# Autodesk Inventor assembly: Front_Train
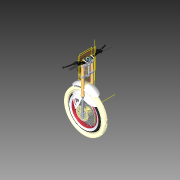
[picture p0: Inventor's stored thumbnail of the model, 180x180]
Saved by Autodesk Inventor 2016 (Build 200138000, 138)
## iProperties
Created: 2015-04-04
Part Number: Front_Train
Document SubType Name: Assembly
Designer: Yann
Author: Yann
## iProperties of the stored document Handlebar.ipt
Created: 2014-11-08
Part Number: Handlebar
Material: Generic
Document SubType Name: Modeling
Designer: Yann
Density: 1 g/cm^3
Appearance: Default
Sending System: SolidWorks 2012
Last Author: Stormtrooper
Last Saved: 2014-11-19
Author: Yann
## Documents named in this file (11)
- **C:\Users\Yann\Documents\GitHub\BIKAIR_CAD\Source\Front_Train\Front_Train.iam*LocalDocs*xOqdabbqfCq0wujc0Oz4mrtfs3b*Handlebar.ipt
- C:\Users\Yann\Documents\GitHub\BIKAIR_CAD\Source\Front_Train\Front_Train.iam
- C:\Users\Yann\Documents\GitHub\BIKAIR_CAD\Source\Front_Train\Fork\Scaled_CR85_Fork.ipt
- C:\Users\Yann\Documents\GitHub\BIKAIR_CAD\Source\Front_Train\Wheel_spokes\Wheel_spokes.iam
- C:\Users\Yann\Documents\GitHub\BIKAIR_CAD\Source\Front_Train\Headlight.iam
- C:\Users\Yann\Documents\GitHub\BIKAIR_CAD\Source\Front_Train\Front_fender.ipt
- C:\Users\Yann\Documents\GitHub\BIKAIR_CAD\Source\Front_Train\Front_fender_without_sides.ipt
- C:\Users\Yann\Documents\GitHub\BIKAIR_CAD\Source\Front_Train\Dashboard\Samsung_S5.ipt
- C:\Users\Yann\Documents\GitHub\BIKAIR_CAD\Source\Front_Train\Brakes\Levers\Manilla.iam
- C:\Users\Yann\Documents\GitHub\BIKAIR_CAD\Source\Front_Train\Handlebar_Grip.ipt
- C:\Users\Yann\Documents\GitHub\BIKAIR_CAD\Source\Front_Train\Handlebar.SLDPRT
## Components (12 placed, 9 different names)
1. Scaled_CR85_Fork:1 — Mate:10, Mate:11, Mate:12, Angle:1
2. Handlebar:2 — Mate:12, Mate:13, Mate:23, Rotational:2, Mate:24, Rotational:3
3. Wheel_spokes:1 [sub-assembly] — Mate:14, Mate:15, Rotational:1
4. Headlight:1 [sub-assembly] — Flush:1, Flush:2
5. Front_fender:1 — Rotational:1
6. Front_fender:2 — Mate:18, Mate:19
7. Front_fender_without_sides:1 — Mate:20, Mate:21
8. Samsung_S5:1 — Mate:22
9. Manilla:1 [sub-assembly] — Mate:23
10. Handlebar_Grip:1 — Rotational:2
11. Manilla:2 [sub-assembly] — Mate:24
12. Handlebar_Grip:2 — Rotational:3
## Relationships (20: Mate 14, RevoluteJoint 3, Flush 2, Angle 1)
- Mate:7
- Mate:10: Scaled_CR85_Fork:1
- Mate:11: Scaled_CR85_Fork:1
- Mate:12: Scaled_CR85_Fork:1 ↔ Handlebar:2
- Mate:13: Handlebar:2
- Mate:14: Wheel_spokes:1
- Mate:15: Wheel_spokes:1
- Flush:1: Headlight:1
- Flush:2: Headlight:1
- Angle:1 (0 deg): Scaled_CR85_Fork:1
- Rotational:1 [RevoluteJoint]: Wheel_spokes:1 ↔ Front_fender:1
- Mate:18 (25 mm): Front_fender:2
- Mate:19: Front_fender:2
- Mate:20 (140 mm): Front_fender_without_sides:1
- Mate:21: Front_fender_without_sides:1
- Mate:22: Samsung_S5:1
- Mate:23: Handlebar:2 ↔ Manilla:1
- Rotational:2 [RevoluteJoint]: Handlebar:2 ↔ Handlebar_Grip:1
- Mate:24: Handlebar:2 ↔ Manilla:2
- Rotational:3 [RevoluteJoint]: Handlebar:2 ↔ Handlebar_Grip:2
